# Autodesk Inventor assembly: A2_PongBoy
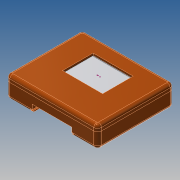
[picture p0: Inventor's stored thumbnail of the model, 180x180]
Saved by Autodesk Inventor 2020.2 (Build 242310000, 310)
## iProperties
Created: 2021-08-29
Part Number: A2_PongBoy
Document SubType Name: Assembly
Designer: Samy Francelet
Author: Samy Francelet
## Documents named in this file (4)
- D:\work\PongBoy\0400_Mechanical\A2_PongBoy.iam
- D:\work\PongBoy\0400_Mechanical\P1_BottomCase.ipt
- D:\work\PongBoy\0400_Mechanical\A1_PCB.iam
- D:\work\PongBoy\0400_Mechanical\A2_TopCase.ipt
## Components (3 placed, 3 different names)
1. P1_BottomCase:1 — Placage:1, Placage:2, Placage:3, Affleurement:1, Affleurement:2, Placage:4
2. A1_PCB:1 [sub-assembly] — Placage:1, Placage:2, Placage:3
3. A2_TopCase:1 — Affleurement:1, Affleurement:2, Placage:4
## Relationships (6: Mate 4, Flush 2)
- Placage:1 [Mate]: P1_BottomCase:1 ↔ A1_PCB:1
- Placage:2 [Mate]: P1_BottomCase:1 ↔ A1_PCB:1
- Placage:3 [Mate]: P1_BottomCase:1 ↔ A1_PCB:1
- Affleurement:1 [Flush]: P1_BottomCase:1 ↔ A2_TopCase:1
- Affleurement:2 [Flush]: P1_BottomCase:1 ↔ A2_TopCase:1
- Placage:4 [Mate]: P1_BottomCase:1 ↔ A2_TopCase:1
